# Autodesk Inventor assembly: hand
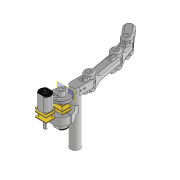
[picture p0: Inventor's stored thumbnail of the model, 180x180]
Saved by Autodesk Inventor 2020.2 (Build 242310000, 310)
## iProperties
Created: 2020-04-08
Part Number: hand
Document SubType Name: Assembly
Designer: Bardo91
thread_hole: 2.500 mm
Author: Bardo91
## Documents named in this file (8)
- D:\programming\bioarm\hardware\hand\hand.iam
- D:\programming\bioarm\hardware\hand\pinky_f1.ipt
- D:\programming\bioarm\hardware\hand\pinky_f2.ipt
- D:\programming\bioarm\hardware\hand\pinky_f3.ipt
- D:\programming\bioarm\hardware\hand\base_hand.ipt
- D:\programming\bioarm\hardware\hand\motor_dc_6v_30rpm.ipt
- D:\programming\bioarm\hardware\hand\finger_thread_lock.ipt
- D:\programming\bioarm\hardware\hand\finger_pulley.ipt
## Components (8 placed, 7 different names)
1. base_hand:1 — Flush:9, Mate:12, Mate:14, Mate:19, Mate:24
2. motor_dc_6v_30rpm:1 — Mate:14, Mate:19, Mate:24, Mate:27, Mate:28, Mate:29
3. motor_dc_6v_30rpm:2
4. finger_thread_lock:1 — Mate:25, Mate:26
5. finger_pulley:1 — Mate:27, Mate:28, Mate:29
6. pinky_f1:1 — Mate:1, Flush:1, Flush:9, Mate:12
7. pinky_f2:1 — Mate:1, Flush:1, Flush:2, Mate:2
8. pinky_f3:1 — Flush:2, Mate:2, Mate:25, Mate:26
## Relationships (14: Mate 11, Flush 3)
- Mate:1: pinky_f1:1 ↔ pinky_f2:1
- Flush:1: pinky_f1:1 ↔ pinky_f2:1
- Flush:2: pinky_f2:1 ↔ pinky_f3:1
- Mate:2: pinky_f2:1 ↔ pinky_f3:1
- Flush:9: base_hand:1 ↔ pinky_f1:1
- Mate:12: base_hand:1 ↔ pinky_f1:1
- Mate:14: base_hand:1 ↔ motor_dc_6v_30rpm:1
- Mate:19: base_hand:1 ↔ motor_dc_6v_30rpm:1
- Mate:24: base_hand:1 ↔ motor_dc_6v_30rpm:1
- Mate:25: finger_thread_lock:1 ↔ pinky_f3:1
- Mate:26 (0.25 mm): finger_thread_lock:1 ↔ pinky_f3:1
- Mate:27: motor_dc_6v_30rpm:1 ↔ finger_pulley:1
- Mate:28 (2 mm): motor_dc_6v_30rpm:1 ↔ finger_pulley:1
- Mate:29: motor_dc_6v_30rpm:1 ↔ finger_pulley:1
## Named parameters: thread_hole = 2.5 mm
